# Autodesk Inventor assembly: DH
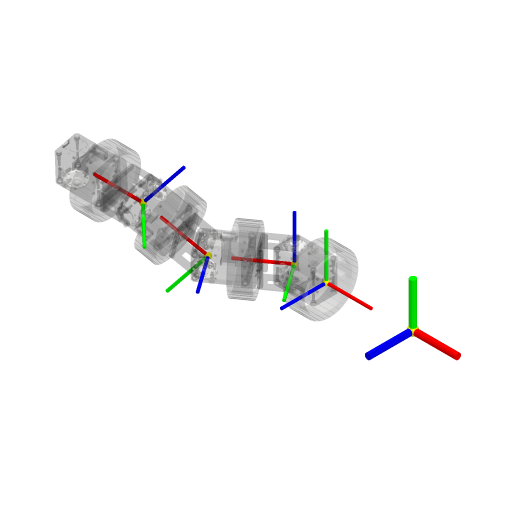
[picture p0: Inventor's stored thumbnail of the model, 512x512]
Saved by Autodesk Inventor 2024 (Build 280153000, 153)
## iProperties
Created: 2023-12-04
Part Number: DH
Document SubType Name: Assembly
Designer: Bong
Author: Bong
## Documents named in this file (6)
- C:\Users\Bong\project\snake_RL\matlab\meshes\Inventor_Reallign\DH\DH.iam
- C:\Users\Bong\project\snake_RL\matlab\meshes\Inventor_Reallign\head\head.iam
- C:\Users\Bong\project\snake_RL\matlab\meshes\Inventor_Reallign\linkA\LinkA.iam
- C:\Users\Bong\project\snake_RL\matlab\meshes\Inventor_Reallign\arrow\arrows2.ipt
- C:\Users\Bong\project\snake_RL\matlab\meshes\Inventor_Reallign\linkB\LinkB.iam
- C:\Users\Bong\project\snake_RL\matlab\meshes\Inventor_Reallign\arrow2\arrows.ipt
## Components (9 placed, 6 different names)
1. Global — 메이트:1
2. Base — 메이트:8, 메이트:9
3. head:1 [sub-assembly] — 플러쉬:1, 플러쉬:2, 플러쉬:3, 회전:1
4. arrows2:1 — 메이트:2, 메이트:3, 플러쉬:4
5. LinkA:1 [sub-assembly] — 회전:1, 회전:2, 메이트:2, 메이트:3, 플러쉬:4
6. arrows2:2 — 메이트:4, 메이트:5
7. LinkB:1 [sub-assembly] — 회전:2, 메이트:4, 메이트:5, 회전:3
8. arrows2:3 — 메이트:6, 메이트:7
9. LinkA:2 [sub-assembly] — 회전:3, 메이트:6, 메이트:7
## Relationships (16: Mate 9, Flush 4, RevoluteJoint 3)
- 플러쉬:1 [Flush]: head:1
- 플러쉬:2 [Flush]: head:1
- 플러쉬:3 [Flush]: head:1
- 회전:1 [RevoluteJoint]: head:1 ↔ LinkA:1
- 회전:2 [RevoluteJoint]: LinkA:1 ↔ LinkB:1
- 메이트:1 [Mate]: Global
- 메이트:2 [Mate]: arrows2:1 ↔ LinkA:1
- 메이트:3 [Mate]: arrows2:1 ↔ LinkA:1
- 플러쉬:4 [Flush]: arrows2:1 ↔ LinkA:1
- 메이트:4 [Mate]: arrows2:2 ↔ LinkB:1
- 메이트:5 [Mate]: arrows2:2 ↔ LinkB:1
- 회전:3 [RevoluteJoint]: LinkB:1 ↔ LinkA:2
- 메이트:6 [Mate]: arrows2:3 ↔ LinkA:2
- 메이트:7 [Mate]: arrows2:3 ↔ LinkA:2
- 메이트:8 [Mate]: Base
- 메이트:9 [Mate]: Base
